# Autodesk Inventor assembly: POM_T5_02
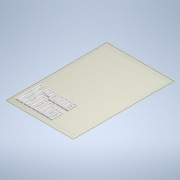
[picture p0: Inventor's stored thumbnail of the model, 180x180]
Saved by Autodesk Inventor 2020 (Build 240168000, 168)
## iProperties
Created: 2021-08-27
Part Number: POM_T5_02
Document SubType Name: Assembly
Designer: Masato
Author: Masato
## Documents named in this file (19)
- C:\Users\Masato\Documents\Inventor\CIT Brains_Inventor\OpenPlatform_ver3_0\cam\POM_T5_02.iam
- C:\Users\Masato\Documents\Inventor\CIT Brains_Inventor\OpenPlatform_ver3_0\cam\Disposable_Board.ipt
- C:\Users\Masato\Documents\Inventor\CIT Brains_Inventor\OpenPlatform_ver3_0\JIG\BackLink_diagonal_jig.ipt
- C:\Users\Masato\Documents\Inventor\CIT Brains_Inventor\OpenPlatform_ver3_0\JIG\Camera_side_frame_jig.ipt
- C:\Users\Masato\Documents\Inventor\CIT Brains_Inventor\OpenPlatform_ver3_0\JIG\Foot_root_block_jig.ipt
- C:\Users\Masato\Documents\Inventor\CIT Brains_Inventor\OpenPlatform_ver3_0\JIG\ForeArm_diagonal_jig_01.ipt
- C:\Users\Masato\Documents\Inventor\CIT Brains_Inventor\OpenPlatform_ver3_0\JIG\ForeArm_diagonal_jig_02.ipt
- C:\Users\Masato\Documents\Inventor\CIT Brains_Inventor\OpenPlatform_ver3_0\JIG\ForeArm_diagonal_jig_03.ipt
- C:\Users\Masato\Documents\Inventor\CIT Brains_Inventor\OpenPlatform_ver3_0\JIG\FrontLink_diagonal_jig.ipt
- C:\Users\Masato\Documents\Inventor\CIT Brains_Inventor\OpenPlatform_ver3_0\JIG\Head_diagonal_jig.ipt
- C:\Users\Masato\Documents\Inventor\CIT Brains_Inventor\OpenPlatform_ver3_0\JIG\Head_horn_frame_jig.ipt
- C:\Users\Masato\Documents\Inventor\CIT Brains_Inventor\OpenPlatform_ver3_0\JIG\Leg_joint_yaw_frame_jig.ipt
- C:\Users\Masato\Documents\Inventor\CIT Brains_Inventor\OpenPlatform_ver3_0\JIG\Shoulder_horn_frame_jig.ipt
- C:\Users\Masato\Documents\Inventor\CIT Brains_Inventor\OpenPlatform_ver3_0\JIG\Trunk_ampit_frame_jig_01.ipt
- C:\Users\Masato\Documents\Inventor\CIT Brains_Inventor\OpenPlatform_ver3_0\JIG\Trunk_ampit_frame_jig_02.ipt
- C:\Users\Masato\Documents\Inventor\CIT Brains_Inventor\OpenPlatform_ver3_0\JIG\Trunk_chest_back_forth_frame_jig_01.ipt
- C:\Users\Masato\Documents\Inventor\CIT Brains_Inventor\OpenPlatform_ver3_0\JIG\Trunk_chest_back_forth_frame_jig_02.ipt
- C:\Users\Masato\Documents\Inventor\CIT Brains_Inventor\OpenPlatform_ver3_0\JIG\Trunk_lower_flank_frame_jig.ipt
- C:\Users\Masato\Documents\Inventor\CIT Brains_Inventor\OpenPlatform_ver3_0\JIG\UpperArm_diagonal_jig.ipt
## Components (18 placed, 18 different names)
1. Disposable_Board:1 — メイト:2, メイト:1, フラッシュ:1, フラッシュ:2, フラッシュ:3, フラッシュ:15
2. BackLink_diagonal_jig:1 — メイト:4, フラッシュ:17, フラッシュ:27, フラッシュ:28
3. Camera_side_frame_jig:1 — メイト:6, フラッシュ:4, メイト:21, メイト:22, フラッシュ:22, メイト:28
4. Foot_root_block_jig:1 — メイト:5, フラッシュ:19, フラッシュ:25, フラッシュ:26
5. ForeArm_diagonal_jig_01:1 — メイト:8, フラッシュ:13, メイト:27, フラッシュ:16
6. ForeArm_diagonal_jig_02:1 — メイト:7, フラッシュ:21, フラッシュ:23, フラッシュ:24
7. ForeArm_diagonal_jig_03:1 — メイト:9, フラッシュ:22, メイト:28, フラッシュ:23
8. FrontLink_diagonal_jig:1 — メイト:10, フラッシュ:5, メイト:22, メイト:23, フラッシュ:21
9. Head_diagonal_jig:1 — メイト:15, フラッシュ:20, フラッシュ:24, フラッシュ:25
10. Head_horn_frame_jig:1 — メイト:16, フラッシュ:18, フラッシュ:26, フラッシュ:27
11. Leg_joint_yaw_frame_jig:1 — メイト:19, フラッシュ:16, フラッシュ:28
12. Shoulder_horn_frame_jig:1 — メイト:11, フラッシュ:10, メイト:26, メイト:27, フラッシュ:17
13. Trunk_ampit_frame_jig_01:1 — メイト:17, フラッシュ:7, メイト:23, メイト:24, フラッシュ:20
14. Trunk_ampit_frame_jig_02:1 — メイト:18, フラッシュ:8, メイト:24, メイト:25, フラッシュ:19
15. Trunk_chest_back_forth_frame_jig_01:1 — メイト:14, フラッシュ:3, フラッシュ:4, フラッシュ:5, フラッシュ:6, フラッシュ:7, フラッシュ:8, フラッシュ:9, フラッシュ:10, フラッシュ:13, メイト:20, フラッシュ:15
16. Trunk_chest_back_forth_frame_jig_02:1 — メイト:12, フラッシュ:9, メイト:25, メイト:26, フラッシュ:18
17. Trunk_lower_flank_frame_jig:1 — メイト:13, フラッシュ:6, メイト:20, メイト:21
18. UpperArm_diagonal_jig:1
## Relationships (52: Mate 27, Flush 25)
- メイト:2 [Mate]: Disposable_Board:1
- メイト:1 [Mate]: Disposable_Board:1
- フラッシュ:1 [Flush]: Disposable_Board:1
- フラッシュ:2 [Flush]: Disposable_Board:1
- メイト:4 [Mate]: BackLink_diagonal_jig:1
- メイト:5 [Mate]: Foot_root_block_jig:1
- メイト:6 [Mate]: Camera_side_frame_jig:1
- メイト:7 [Mate]: ForeArm_diagonal_jig_02:1
- メイト:8 [Mate]: ForeArm_diagonal_jig_01:1
- メイト:9 [Mate]: ForeArm_diagonal_jig_03:1
- メイト:10 [Mate]: FrontLink_diagonal_jig:1
- メイト:11 [Mate]: Shoulder_horn_frame_jig:1
- メイト:12 [Mate]: Trunk_chest_back_forth_frame_jig_02:1
- メイト:13 [Mate]: Trunk_lower_flank_frame_jig:1
- メイト:14 [Mate]: Trunk_chest_back_forth_frame_jig_01:1
- メイト:15 [Mate]: Head_diagonal_jig:1
- メイト:16 [Mate]: Head_horn_frame_jig:1
- メイト:17 [Mate]: Trunk_ampit_frame_jig_01:1
- メイト:18 [Mate]: Trunk_ampit_frame_jig_02:1
- メイト:19 [Mate]: Leg_joint_yaw_frame_jig:1
- フラッシュ:3 [Flush] (3 mm): Disposable_Board:1 ↔ Trunk_chest_back_forth_frame_jig_01:1
- フラッシュ:4 [Flush]: Camera_side_frame_jig:1 ↔ Trunk_chest_back_forth_frame_jig_01:1
- フラッシュ:5 [Flush]: FrontLink_diagonal_jig:1 ↔ Trunk_chest_back_forth_frame_jig_01:1
- フラッシュ:6 [Flush]: Trunk_chest_back_forth_frame_jig_01:1 ↔ Trunk_lower_flank_frame_jig:1
- フラッシュ:7 [Flush]: Trunk_ampit_frame_jig_01:1 ↔ Trunk_chest_back_forth_frame_jig_01:1
- フラッシュ:8 [Flush]: Trunk_ampit_frame_jig_02:1 ↔ Trunk_chest_back_forth_frame_jig_01:1
- フラッシュ:9 [Flush]: Trunk_chest_back_forth_frame_jig_01:1 ↔ Trunk_chest_back_forth_frame_jig_02:1
- フラッシュ:10 [Flush]: Shoulder_horn_frame_jig:1 ↔ Trunk_chest_back_forth_frame_jig_01:1
- フラッシュ:13 [Flush]: ForeArm_diagonal_jig_01:1 ↔ Trunk_chest_back_forth_frame_jig_01:1
- メイト:20 [Mate] (2.5 mm): Trunk_chest_back_forth_frame_jig_01:1 ↔ Trunk_lower_flank_frame_jig:1
- メイト:21 [Mate] (2.5 mm): Camera_side_frame_jig:1 ↔ Trunk_lower_flank_frame_jig:1
- メイト:22 [Mate] (2.5 mm): Camera_side_frame_jig:1 ↔ FrontLink_diagonal_jig:1
- メイト:23 [Mate] (2.5 mm): FrontLink_diagonal_jig:1 ↔ Trunk_ampit_frame_jig_01:1
- メイト:24 [Mate] (2.5 mm): Trunk_ampit_frame_jig_01:1 ↔ Trunk_ampit_frame_jig_02:1
- メイト:25 [Mate] (2.5 mm): Trunk_ampit_frame_jig_02:1 ↔ Trunk_chest_back_forth_frame_jig_02:1
- メイト:26 [Mate] (2.5 mm): Shoulder_horn_frame_jig:1 ↔ Trunk_chest_back_forth_frame_jig_02:1
- メイト:27 [Mate] (2.5 mm): ForeArm_diagonal_jig_01:1 ↔ Shoulder_horn_frame_jig:1
- フラッシュ:15 [Flush] (3 mm): Disposable_Board:1 ↔ Trunk_chest_back_forth_frame_jig_01:1
- フラッシュ:16 [Flush]: ForeArm_diagonal_jig_01:1 ↔ Leg_joint_yaw_frame_jig:1
- フラッシュ:17 [Flush]: BackLink_diagonal_jig:1 ↔ Shoulder_horn_frame_jig:1
- フラッシュ:18 [Flush]: Head_horn_frame_jig:1 ↔ Trunk_chest_back_forth_frame_jig_02:1
- フラッシュ:19 [Flush]: Foot_root_block_jig:1 ↔ Trunk_ampit_frame_jig_02:1
- フラッシュ:20 [Flush]: Head_diagonal_jig:1 ↔ Trunk_ampit_frame_jig_01:1
- フラッシュ:21 [Flush]: ForeArm_diagonal_jig_02:1 ↔ FrontLink_diagonal_jig:1
- フラッシュ:22 [Flush]: Camera_side_frame_jig:1 ↔ ForeArm_diagonal_jig_03:1
- メイト:28 [Mate] (2.5 mm): Camera_side_frame_jig:1 ↔ ForeArm_diagonal_jig_03:1
- フラッシュ:23 [Flush]: ForeArm_diagonal_jig_02:1 ↔ ForeArm_diagonal_jig_03:1
- フラッシュ:24 [Flush]: ForeArm_diagonal_jig_02:1 ↔ Head_diagonal_jig:1
- フラッシュ:25 [Flush]: Foot_root_block_jig:1 ↔ Head_diagonal_jig:1
- フラッシュ:26 [Flush]: Foot_root_block_jig:1 ↔ Head_horn_frame_jig:1
- フラッシュ:27 [Flush]: BackLink_diagonal_jig:1 ↔ Head_horn_frame_jig:1
- フラッシュ:28 [Flush]: BackLink_diagonal_jig:1 ↔ Leg_joint_yaw_frame_jig:1
